# Autodesk Inventor assembly: Elevator Base
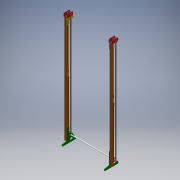
[picture p0: Inventor's stored thumbnail of the model, 180x180]
Saved by Autodesk Inventor 2017 SP1 (Build 210196100, 196)
## iProperties
Created: 2018-01-18
Part Number: Elevator Base
Document SubType Name: Assembly
Designer: Ben
Mass: 9979.66 g
Surface Area: 70095.8 cm^2
Volume: 103427 cm^3
Density: 0.0964899 g/cm^3
Author: Ben
## Documents named in this file (9)
- C:\Users\Ben\Desktop\Projects\2018 Robot\Cube Lift\Elevator Base.iam
- C:\Users\Ben\Desktop\Projects\2018 Robot\Cube Lift\Rail.ipt
- C:\Users\Ben\Desktop\Projects\2018 Robot\Cube Lift\support plate 2.ipt
- C:\Users\Ben\Desktop\Projects\2018 Robot\Cube Lift\top pully bracket.ipt
- C:\Users\Ben\Desktop\Projects\2018 Robot\Cube Lift\pulley XL 1in.ipt
- C:\Users\Ben\Desktop\Projects\2018 Robot\Cube Lift\pulley XL 1.375in 2.ipt
- C:\Users\Ben\Desktop\Projects\2018 Robot\Cube Lift\first stage belt.ipt
- C:\Users\Ben\Desktop\Projects\2018 Robot\Cube Lift\upper anchor.ipt
- C:\Users\Ben\Desktop\Projects\2018 Robot\Cube Lift\driveshaft.ipt
## Components (15 placed, 8 different names)
1. Rail:1 — Mate:30, Flush:29, Mate:39, Flush:30, Angle:2, Flush:33, Mate:44, Flush:43, Flush:53
2. support plate 2:1 — Mate:30, Insert:8, Flush:43, Flush:56, Mate:103
3. top pully bracket:1 — Flush:29, Mate:39, Flush:30, Mate:40, Flush:31, Mate:65
4. pulley XL 1in:1 — Insert:8, Insert:9
5. pulley XL 1.375in 2:1 — Mate:40, Flush:31
6. first stage belt:1 — Insert:9, Angle:2, Flush:65
7. upper anchor:1 — Flush:33, Mate:44, Mate:65
8. driveshaft:1 — Flush:52, Mate:103, Mate:104
9. support plate 2:2 — Mate:79, Flush:55, Flush:56, Insert:25, Mate:104
10. Rail:5 — Flush:53, Mate:79, Flush:55, Mate:94, Flush:61, Flush:62, Mate:99
11. pulley XL 1in:2 — Insert:25, Insert:30
12. top pully bracket:2 — Mate:94, Flush:61, Flush:62, Mate:95, Mate:96, Mate:100
13. pulley XL 1.375in 2:2 — Mate:95, Mate:96
14. upper anchor:2 — Mate:99, Mate:100
15. first stage belt:2 — Insert:30, Flush:65
## Relationships (30: Mate 13, Flush 12, Insert 4, Angle 1)
- Mate:30: Rail:1 ↔ support plate 2:1
- Flush:29 (-1.5875 mm): Rail:1 ↔ top pully bracket:1
- Mate:39: Rail:1 ↔ top pully bracket:1
- Flush:30 (6.35 mm): Rail:1 ↔ top pully bracket:1
- Insert:8 (4.7625 mm): support plate 2:1 ↔ pulley XL 1in:1
- Mate:40: top pully bracket:1 ↔ pulley XL 1.375in 2:1
- Flush:31: top pully bracket:1 ↔ pulley XL 1.375in 2:1
- Insert:9 (1.5875 mm): pulley XL 1in:1 ↔ first stage belt:1
- Angle:2 (0 deg): Rail:1 ↔ first stage belt:1
- Flush:33: Rail:1 ↔ upper anchor:1
- Mate:44: Rail:1 ↔ upper anchor:1
- Flush:43: Rail:1 ↔ support plate 2:1
- Mate:65: top pully bracket:1 ↔ upper anchor:1
- Flush:52: driveshaft:1
- Flush:53: Rail:1 ↔ Rail:5
- Mate:79: support plate 2:2 ↔ Rail:5
- Flush:55: support plate 2:2 ↔ Rail:5
- Flush:56: support plate 2:1 ↔ support plate 2:2
- Insert:25 (4.7625 mm): support plate 2:2 ↔ pulley XL 1in:2
- Mate:94: Rail:5 ↔ top pully bracket:2
- Flush:61 (-1.5875 mm): Rail:5 ↔ top pully bracket:2
- Flush:62 (-6.35 mm): Rail:5 ↔ top pully bracket:2
- Mate:95 (6.35 mm): top pully bracket:2 ↔ pulley XL 1.375in 2:2
- Mate:96: top pully bracket:2 ↔ pulley XL 1.375in 2:2
- Mate:99: Rail:5 ↔ upper anchor:2
- Mate:100: top pully bracket:2 ↔ upper anchor:2
- Insert:30 (1.5875 mm): pulley XL 1in:2 ↔ first stage belt:2
- Flush:65: first stage belt:1 ↔ first stage belt:2
- Mate:103: support plate 2:1 ↔ driveshaft:1
- Mate:104: driveshaft:1 ↔ support plate 2:2
